# Autodesk Inventor assembly: 3-15
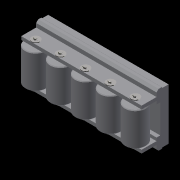
[picture p0: Inventor's stored thumbnail of the model, 180x180]
Saved by Autodesk Inventor 2017 (Build 210142000, 142)
## iProperties
Part Number: 3-15
Material: 一般
Document SubType Name: Assembly
Designer: r0909
Author: r0909
## Documents named in this file (8)
- C:\Users\r0909\Desktop\inventor\3-15.iam
- C:\Users\r0909\Desktop\inventor\3-11.ipt
- C:\Users\r0909\Desktop\inventor\3-12.ipt
- C:\Users\r0909\Desktop\inventor\3-13.ipt
- C:\Users\r0909\Desktop\inventor\3-14.ipt
- C:\Users\r0909\Desktop\inventor\3-15.1.ipt
- C:\Users\r0909\Desktop\inventor\3-15.2.ipt
- C:\Users\r0909\Documents\Inventor\Content Center Files\R2017\zh-TW\CNS 5050\CNS 5050 - A - 11 40.ipt
## Components (40 placed, 7 different names)
1. 3-11:1 — 貼合:12, 貼合:13, 齊平:5, 貼合:30, 貼合:46
2. 3-12:1 — 貼合:8, 貼合:9, 齊平:3, 貼合:12, 貼合:14, 貼合:15, 貼合:16, 貼合:17, 貼合:31, 角度:2
3. 3-13:1 — 貼合:2, 貼合:3, 貼合:4, 貼合:10, 貼合:11, 齊平:4
4. 3-14:1 — 齊平:2, 貼合:1, 貼合:2, 貼合:3, 貼合:4, 貼合:5, 貼合:6, 貼合:7, 貼合:13, 貼合:18, 相切:1, 角度:1, 貼合:19, 貼合:20, 貼合:21, 貼合:22, 貼合:23, 貼合:24, 貼合:25, 貼合:26, 貼合:27
5. 3-13:2 — 貼合:5, 貼合:6, 貼合:7, 貼合:8, 貼合:9, 齊平:3
6. 3-12:2 — 貼合:10, 貼合:11, 齊平:4, 貼合:47, 角度:3
7. 3-11:2 — 貼合:14, 齊平:5, 齊平:6, 貼合:40, 貼合:56
8. 3-11:3 — 貼合:15, 齊平:6, 齊平:7, 貼合:41, 貼合:57
9. 3-11:4 — 貼合:16, 齊平:7, 齊平:8, 貼合:42, 貼合:58
10. 3-11:5 — 貼合:17, 齊平:8, 貼合:43, 貼合:59
11. 3-15.1:1 — 貼合:18, 相切:1, 角度:1, 齊平:9
12. 3-15.1:2 — 貼合:27, 齊平:17
13. 3-15.1:3 — 貼合:26, 齊平:16, 齊平:17
14. 3-15.1:4 — 貼合:25, 齊平:15, 齊平:16
15. 3-15.1:5 — 貼合:24, 齊平:14, 齊平:15
16. 3-15.1:6 — 貼合:23, 齊平:13, 齊平:14
17. 3-15.1:7 — 貼合:22, 齊平:12, 齊平:13
18. 3-15.1:8 — 貼合:21, 齊平:11, 齊平:12
19. 3-15.1:9 — 貼合:20, 齊平:10, 齊平:11
20. 3-15.1:10 — 貼合:19, 齊平:9, 齊平:10
21. 3-15.2:1 — 貼合:28, 貼合:29, 貼合:30, 角度:2, 齊平:21
22. CNS 5050 A - 11:1 — 貼合:28, 貼合:29, 貼合:31
23. 3-15.2:2 — 貼合:40, 齊平:20, 齊平:21
24. CNS 5050 A - 11:2
25. 3-15.2:3 — 貼合:41, 齊平:19, 齊平:20
26. CNS 5050 A - 11:3
27. 3-15.2:4 — 貼合:42, 齊平:18, 齊平:19
28. CNS 5050 A - 11:4
29. 3-15.2:5 — 貼合:43, 齊平:18
30. CNS 5050 A - 11:5
31. 3-15.2:6 — 貼合:46, 角度:3, 齊平:25
32. CNS 5050 A - 11:6 — 貼合:47
33. 3-15.2:7 — 貼合:56, 齊平:24, 齊平:25
34. CNS 5050 A - 11:7
35. 3-15.2:8 — 貼合:57, 齊平:23, 齊平:24
36. CNS 5050 A - 11:8
37. 3-15.2:9 — 貼合:58, 齊平:22, 齊平:23
38. CNS 5050 A - 11:9
39. 3-15.2:10 — 貼合:59, 齊平:22
40. CNS 5050 A - 11:10
## Relationships (87: Mate 59, Flush 24, Angle 3, Tangent 1)
- 齊平:2 [Flush]: 3-14:1
- 貼合:1 [Mate]: 3-14:1
- 貼合:2 [Mate]: 3-13:1 ↔ 3-14:1
- 貼合:3 [Mate]: 3-13:1 ↔ 3-14:1
- 貼合:4 [Mate]: 3-13:1 ↔ 3-14:1
- 貼合:5 [Mate]: 3-14:1 ↔ 3-13:2
- 貼合:6 [Mate]: 3-14:1 ↔ 3-13:2
- 貼合:7 [Mate]: 3-14:1 ↔ 3-13:2
- 貼合:8 [Mate]: 3-12:1 ↔ 3-13:2
- 貼合:9 [Mate]: 3-12:1 ↔ 3-13:2
- 齊平:3 [Flush]: 3-12:1 ↔ 3-13:2
- 貼合:10 [Mate]: 3-13:1 ↔ 3-12:2
- 貼合:11 [Mate]: 3-13:1 ↔ 3-12:2
- 齊平:4 [Flush]: 3-13:1 ↔ 3-12:2
- 貼合:12 [Mate]: 3-11:1 ↔ 3-12:1
- 貼合:13 [Mate]: 3-11:1 ↔ 3-14:1
- 貼合:14 [Mate]: 3-12:1 ↔ 3-11:2
- 貼合:15 [Mate]: 3-12:1 ↔ 3-11:3
- 貼合:16 [Mate]: 3-12:1 ↔ 3-11:4
- 貼合:17 [Mate]: 3-12:1 ↔ 3-11:5
- 齊平:5 [Flush]: 3-11:1 ↔ 3-11:2
- 齊平:6 [Flush]: 3-11:2 ↔ 3-11:3
- 齊平:7 [Flush]: 3-11:3 ↔ 3-11:4
- 齊平:8 [Flush]: 3-11:4 ↔ 3-11:5
- 貼合:18 [Mate]: 3-14:1 ↔ 3-15.1:1
- 相切:1 [Tangent]: 3-14:1 ↔ 3-15.1:1
- 角度:1 [Angle] (0 deg): 3-14:1 ↔ 3-15.1:1
- 貼合:19 [Mate]: 3-14:1 ↔ 3-15.1:10
- 貼合:20 [Mate]: 3-14:1 ↔ 3-15.1:9
- 貼合:21 [Mate]: 3-14:1 ↔ 3-15.1:8
- 貼合:22 [Mate]: 3-14:1 ↔ 3-15.1:7
- 貼合:23 [Mate]: 3-14:1 ↔ 3-15.1:6
- 貼合:24 [Mate]: 3-14:1 ↔ 3-15.1:5
- 貼合:25 [Mate]: 3-14:1 ↔ 3-15.1:4
- 貼合:26 [Mate]: 3-14:1 ↔ 3-15.1:3
- 貼合:27 [Mate]: 3-14:1 ↔ 3-15.1:2
- 齊平:9 [Flush]: 3-15.1:1 ↔ 3-15.1:10
- 齊平:10 [Flush]: 3-15.1:9 ↔ 3-15.1:10
- 齊平:11 [Flush]: 3-15.1:8 ↔ 3-15.1:9
- 齊平:12 [Flush]: 3-15.1:7 ↔ 3-15.1:8
- 齊平:13 [Flush]: 3-15.1:6 ↔ 3-15.1:7
- 齊平:14 [Flush]: 3-15.1:5 ↔ 3-15.1:6
- 齊平:15 [Flush]: 3-15.1:4 ↔ 3-15.1:5
- 齊平:16 [Flush]: 3-15.1:3 ↔ 3-15.1:4
- 齊平:17 [Flush]: 3-15.1:2 ↔ 3-15.1:3
- 貼合:28 [Mate]: 3-15.2:1 ↔ CNS 5050 A - 11:1
- 貼合:29 [Mate]: 3-15.2:1 ↔ CNS 5050 A - 11:1
- 貼合:30 [Mate]: 3-11:1 ↔ 3-15.2:1
- 貼合:31 [Mate]: 3-12:1 ↔ CNS 5050 A - 11:1
- 角度:2 [Angle] (0 deg): 3-12:1 ↔ 3-15.2:1
- [Mate]: 3-15.2:2 ↔ CNS 5050 A - 11:2
- [Mate]: 3-15.2:2 ↔ CNS 5050 A - 11:2
- [Mate]: 3-15.2:3 ↔ CNS 5050 A - 11:3
- [Mate]: 3-15.2:3 ↔ CNS 5050 A - 11:3
- [Mate]: 3-15.2:4 ↔ CNS 5050 A - 11:4
- [Mate]: 3-15.2:4 ↔ CNS 5050 A - 11:4
- [Mate]: 3-15.2:5 ↔ CNS 5050 A - 11:5
- [Mate]: 3-15.2:5 ↔ CNS 5050 A - 11:5
- 貼合:40 [Mate]: 3-11:2 ↔ 3-15.2:2
- 貼合:41 [Mate]: 3-11:3 ↔ 3-15.2:3
- 貼合:42 [Mate]: 3-11:4 ↔ 3-15.2:4
- 貼合:43 [Mate]: 3-11:5 ↔ 3-15.2:5
- 齊平:18 [Flush]: 3-15.2:4 ↔ 3-15.2:5
- 齊平:19 [Flush]: 3-15.2:3 ↔ 3-15.2:4
- 齊平:20 [Flush]: 3-15.2:2 ↔ 3-15.2:3
- 齊平:21 [Flush]: 3-15.2:1 ↔ 3-15.2:2
- [Mate]: 3-15.2:6 ↔ CNS 5050 A - 11:6
- [Mate]: 3-15.2:6 ↔ CNS 5050 A - 11:6
- 貼合:46 [Mate]: 3-11:1 ↔ 3-15.2:6
- 貼合:47 [Mate]: 3-12:2 ↔ CNS 5050 A - 11:6
- 角度:3 [Angle] (0 deg): 3-12:2 ↔ 3-15.2:6
- [Mate]: 3-15.2:7 ↔ CNS 5050 A - 11:7
- [Mate]: 3-15.2:7 ↔ CNS 5050 A - 11:7
- [Mate]: 3-15.2:8 ↔ CNS 5050 A - 11:8
- [Mate]: 3-15.2:8 ↔ CNS 5050 A - 11:8
- [Mate]: 3-15.2:9 ↔ CNS 5050 A - 11:9
- [Mate]: 3-15.2:9 ↔ CNS 5050 A - 11:9
- [Mate]: 3-15.2:10 ↔ CNS 5050 A - 11:10
- [Mate]: 3-15.2:10 ↔ CNS 5050 A - 11:10
- 貼合:56 [Mate]: 3-11:2 ↔ 3-15.2:7
- 貼合:57 [Mate]: 3-11:3 ↔ 3-15.2:8
- 貼合:58 [Mate]: 3-11:4 ↔ 3-15.2:9
- 貼合:59 [Mate]: 3-11:5 ↔ 3-15.2:10
- 齊平:22 [Flush]: 3-15.2:9 ↔ 3-15.2:10
- 齊平:23 [Flush]: 3-15.2:8 ↔ 3-15.2:9
- 齊平:24 [Flush]: 3-15.2:7 ↔ 3-15.2:8
- 齊平:25 [Flush]: 3-15.2:6 ↔ 3-15.2:7
## Named parameters: d53_d48 = 0 mm, d54_d49 = 0 mm, d55_d48 = 0 mm, d56_d49 = 0 mm, d57_d48 = 0 mm, d58_d49 = 0 mm, d59_d48 = 0 mm, d60_d49 = 0 mm, d69_d48 = 0 mm, d70_d49 = 0 mm, d74_d69_d48 = 0 mm, d75_d70_d49 = 0 mm, d76_d69_d48 = 0 mm, d77_d70_d49 = 0 mm, d78_d69_d48 = 0 mm, d79_d70_d49 = 0 mm, d80_d69_d48 = 0 mm, d81_d70_d49 = 0 mm
